# Autodesk Inventor assembly: DribblerUnit
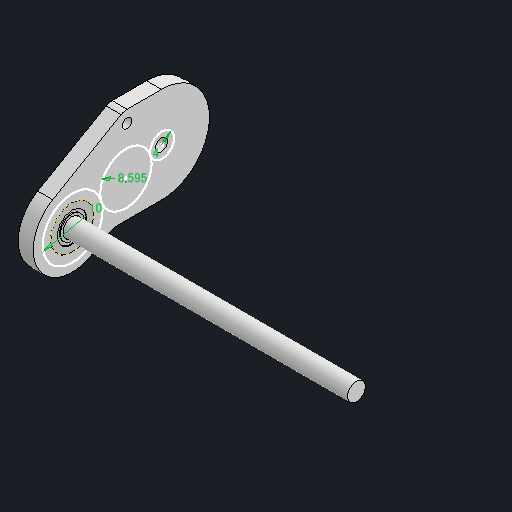
[picture p0: Inventor's stored thumbnail of the model, 512x512]
Saved by Autodesk Inventor 2024.2 (Build 282272000, 272)
## iProperties
Created: 2023-12-27
Part Number: DribblerUnit
Document SubType Name: Assembly
Designer: Hanaoka
Author: Hanaoka
## Documents named in this file (4)
- G:\共有ドライブ\reRo\05_個人\hanaoka\inventor\DribblerUnit\DribblerUnit.iam
- G:\共有ドライブ\reRo\05_個人\hanaoka\inventor\HandleUnit\GearCover.ipt
- G:\共有ドライブ\reRo\05_個人\hanaoka\inventor\DribblerUnit\Shaft.ipt
- G:\共有ドライブ\reRo\05_個人\hanaoka\inventor\DribblerUnit\Bearing_C-FL673ZZ.ipt
## Components (3 placed, 3 different names)
1. GearCover:1 — 挿入:1
2. Shaft:1 — 挿入:2
3. Bearing_C-FL673ZZ:1 — 挿入:1, 挿入:2
## Relationships (2: Insert 2)
- 挿入:1 [Insert]: GearCover:1 ↔ Bearing_C-FL673ZZ:1
- 挿入:2 [Insert]: Shaft:1 ↔ Bearing_C-FL673ZZ:1
